# Autodesk Inventor assembly: Intake New Robot
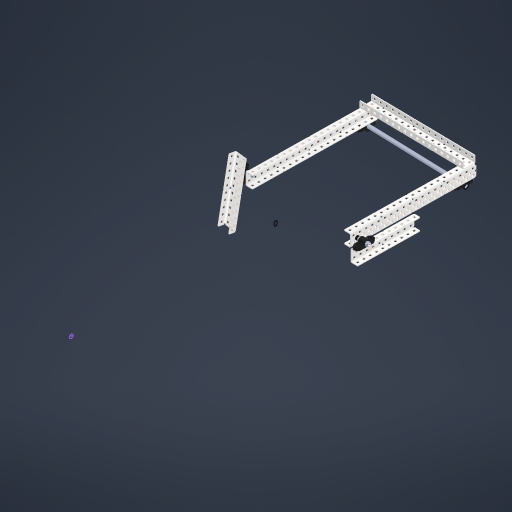
[picture p0: Inventor's stored thumbnail of the model, 512x512]
Saved by Autodesk Inventor 2023 (Build 270158000, 158)
## iProperties
Created: 2023-11-27
Part Number: Intake New Robot
Document SubType Name: Assembly
Designer: Robodox
Author: Robodox
## Documents named in this file (17)
- C:\Users\diego\OneDrive\Documents\GitHub\2023-599Z\BBotCAD\Intake New Robot.iam
- C:\Users\Robodox\Downloads\High Strength Pillow Block Bearing (276-8383).ipt
- C:\Users\diego\OneDrive\Documents\GitHub\2023-599Z\BBotCAD\VEX-CAD-Inventor-1.4.0\Structure\C Channel\Aluminum 1x2x1\Alu C 1x2x1x10.ipt
- C:\Users\diego\OneDrive\Documents\GitHub\2023-599Z\BBotCAD\VEX-CAD-Inventor-1.4.0\Structure\Hardware\Screw Steel - Star\SScrew Star Smooth 1.000.ipt
- C:\Users\Robodox\Documents\GitHub\2023-599Z\BBotCAD\VEX-CAD-Inventor-1.4.0\Structure\Hardware\Screw Steel - Star.ipt
- C:\Users\diego\OneDrive\Documents\GitHub\2023-599Z\BBotCAD\VEX-CAD-Inventor-1.4.0\Structure\Hardware\Nut Nylock.ipt
- C:\Users\diego\OneDrive\Documents\GitHub\2023-599Z\BBotCAD\VEX-CAD-Inventor-1.4.0\Structure\Hardware\Nut Keps.ipt
- C:\Users\diego\OneDrive\Documents\GitHub\2023-599Z\BBotCAD\VEX-CAD-Inventor-1.4.0\Motion\Spacers\Spacer Plastic\PSpacer 4.6.ipt
- C:\Users\Robodox\Documents\GitHub\2023-599Z\BBotCAD\VEX-CAD-Inventor-1.4.0\Motion\Spacers\Spacer Plastic.ipt
- C:\Users\diego\OneDrive\Documents\GitHub\2023-599Z\BBotCAD\VEX-CAD-Inventor-1.4.0\Structure\C Channel\Aluminum 1x2x1\Alu C 1x2x1x20.ipt
- C:\Users\diego\OneDrive\Documents\GitHub\2023-599Z\BBotCAD\VEX-CAD-Inventor-1.4.0\Structure\C Channel\Aluminum 1x2x1\Alu C 1x2x1x1.ipt
- C:\Users\diego\OneDrive\Documents\GitHub\2023-599Z\BBotCAD\VEX-CAD-Inventor-1.4.0\Structure\C Channel\Aluminum 1x2x1\Alu C 1x2x1x17.ipt
- C:\Users\diego\OneDrive\Documents\GitHub\2023-599Z\BBotCAD\VEX-CAD-Inventor-1.4.0\Motion\Shaft HS\HS Pillow Bearing Block.ipt
- C:\Users\diego\OneDrive\Documents\GitHub\2023-599Z\BBotCAD\VEX-CAD-Inventor-1.4.0\Motion\Shaft HS\Shaft HS.ipt
- C:\Users\diego\OneDrive\Documents\GitHub\2023-599Z\BBotCAD\VEX-CAD-Inventor-1.4.0\Motion\Shaft HS\Shaft HS\Shaft HS 9.0 in.ipt
- C:\Users\diego\OneDrive\Documents\GitHub\2023-599Z\BBotCAD\VEX-CAD-Inventor-1.4.0\Motion\Shaft HS\HS Spacer\HSpacer .0625.ipt
- C:\Users\diego\OneDrive\Documents\GitHub\2023-599Z\BBotCAD\VEX-CAD-Inventor-1.4.0\Motion\Shaft HS\HS Spacer.ipt
## Components (25 placed, 12 different names)
1. High Strength Pillow Block Bearing (276-8383):1
2. Alu C 1x2x1x10:1 — Insert:24, Insert:25
3. Alu C 1x2x1x10:2 — Insert:6, Insert:26, Insert:27
4. SScrew Star Smooth 1.000:1 — Insert:5, Insert:21, Insert:23
5. Nut Nylock:1 — Insert:23
6. Nut Nylock:2 — Insert:15
7. Nut Keps:2 — Insert:13, Mate:5
8. PSpacer 4.6:1 — Insert:21, Insert:22
9. Alu C 1x2x1x20:2 — Insert:5, Insert:16, Insert:17, Insert:28, Insert:30, Insert:32, Insert:33
10. High Strength Pillow Block Bearing (276-8383):2 — Insert:6, Mate:3
11. Nut Keps:3 — Insert:22, Mate:6
12. Alu C 1x2x1x1:1 — Mate:3, Insert:14, Mate:4
13. Alu C 1x2x1x20:4 — Insert:11, Insert:12, Insert:18, Insert:19, Insert:20, Insert:29, Insert:31, Insert:34
14. SScrew Star Smooth 1.000:2 — Insert:11, Insert:14, Insert:15
15. PSpacer 4.6:2 — Insert:12, Insert:13
16. High Strength Pillow Block Bearing (276-8383):3 — Insert:16, Insert:17
17. High Strength Pillow Block Bearing (276-8383):4 — Insert:18, Insert:19
18. Alu C 1x2x1x17:2 — Insert:20, Insert:28, Insert:31, Insert:32
19. HS Pillow Bearing Block:1 — Insert:26, Insert:27, Mate:4, Mate:5
20. HS Pillow Bearing Block:2 — Insert:24, Insert:25, Mate:6
21. HS Pillow Bearing Block:3 — Insert:30, Mate:13, Insert:33
22. HS Pillow Bearing Block:4 — Insert:29, Mate:10, Mate:11, Insert:34
23. Shaft HS 9.0 in:2 — Mate:7, Mate:8, Mate:9, Mate:12
24. HSpacer .0625:1 — Mate:7, Mate:8, Mate:9, Mate:10, Mate:11
25. HSpacer .0625:2 — Mate:12, Mate:13
## Relationships (37: Insert 26, Mate 11)
- Insert:5: SScrew Star Smooth 1.000:1 ↔ Alu C 1x2x1x20:2
- Insert:6: Alu C 1x2x1x10:2 ↔ High Strength Pillow Block Bearing (276-8383):2
- Insert:11: Alu C 1x2x1x20:4 ↔ SScrew Star Smooth 1.000:2
- Insert:12: Alu C 1x2x1x20:4 ↔ PSpacer 4.6:2
- Insert:13: Nut Keps:2 ↔ PSpacer 4.6:2
- Mate:3: High Strength Pillow Block Bearing (276-8383):2 ↔ Alu C 1x2x1x1:1
- Insert:14 (-15.494 mm): Alu C 1x2x1x1:1 ↔ SScrew Star Smooth 1.000:2
- Insert:15 (-3.048 mm): Nut Nylock:2 ↔ SScrew Star Smooth 1.000:2
- Insert:16: Alu C 1x2x1x20:2 ↔ High Strength Pillow Block Bearing (276-8383):3
- Insert:17: Alu C 1x2x1x20:2 ↔ High Strength Pillow Block Bearing (276-8383):3
- Insert:18: Alu C 1x2x1x20:4 ↔ High Strength Pillow Block Bearing (276-8383):4
- Insert:19: Alu C 1x2x1x20:4 ↔ High Strength Pillow Block Bearing (276-8383):4
- Insert:20: Alu C 1x2x1x20:4 ↔ Alu C 1x2x1x17:2
- Insert:21 (-23.8252 mm): SScrew Star Smooth 1.000:1 ↔ PSpacer 4.6:1
- Insert:22: PSpacer 4.6:1 ↔ Nut Keps:3
- Insert:23 (-3.048 mm): SScrew Star Smooth 1.000:1 ↔ Nut Nylock:1
- Insert:24: Alu C 1x2x1x10:1 ↔ HS Pillow Bearing Block:2
- Insert:25: Alu C 1x2x1x10:1 ↔ HS Pillow Bearing Block:2
- Insert:26: Alu C 1x2x1x10:2 ↔ HS Pillow Bearing Block:1
- Insert:27: Alu C 1x2x1x10:2 ↔ HS Pillow Bearing Block:1
- Mate:4: Alu C 1x2x1x1:1 ↔ HS Pillow Bearing Block:1
- Mate:5: Nut Keps:2 ↔ HS Pillow Bearing Block:1
- Mate:6: Nut Keps:3 ↔ HS Pillow Bearing Block:2
- Insert:28: Alu C 1x2x1x20:2 ↔ Alu C 1x2x1x17:2
- Insert:29: Alu C 1x2x1x20:4 ↔ HS Pillow Bearing Block:4
- Insert:30: Alu C 1x2x1x20:2 ↔ HS Pillow Bearing Block:3
- Mate:7: Shaft HS 9.0 in:2 ↔ HSpacer .0625:1
- Mate:8: Shaft HS 9.0 in:2 ↔ HSpacer .0625:1
- Mate:9: Shaft HS 9.0 in:2 ↔ HSpacer .0625:1
- Mate:10: HS Pillow Bearing Block:4 ↔ HSpacer .0625:1
- Mate:11: HS Pillow Bearing Block:4 ↔ HSpacer .0625:1
- Mate:12: Shaft HS 9.0 in:2 ↔ HSpacer .0625:2
- Mate:13: HS Pillow Bearing Block:3 ↔ HSpacer .0625:2
- Insert:31: Alu C 1x2x1x20:4 ↔ Alu C 1x2x1x17:2
- Insert:32: Alu C 1x2x1x20:2 ↔ Alu C 1x2x1x17:2
- Insert:33: Alu C 1x2x1x20:2 ↔ HS Pillow Bearing Block:3
- Insert:34: Alu C 1x2x1x20:4 ↔ HS Pillow Bearing Block:4
